# Autodesk Inventor assembly: Assembly1
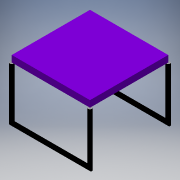
[picture p0: Inventor's stored thumbnail of the model, 180x180]
Saved by Autodesk Inventor 2016 (Build 200138000, 138)
## iProperties
Created: 2017-12-15
Part Number: Assembly1
Document SubType Name: Assembly
Designer: sun01147
Author: sun01147
## Documents named in this file (3)
- E:\IED7_SunT\IED7_Practice\Assembly1.iam
- E:\IED7_SunT\IED7_Practice\Leg.ipt
- E:\IED7_SunT\IED7_Practice\Table_Top.ipt
## Components (3 placed, 2 different names)
1. Table_Top:1 — Mate:1, Mate:2, Mate:3, Mate:4
2. Leg:1 — Mate:1, Mate:4
3. Leg:2 — Mate:2, Mate:3
## Relationships (4: Mate 4)
- Mate:1: Table_Top:1 ↔ Leg:1
- Mate:2: Table_Top:1 ↔ Leg:2
- Mate:3: Table_Top:1 ↔ Leg:2
- Mate:4: Table_Top:1 ↔ Leg:1
